# Autodesk Inventor assembly: 마지막센서
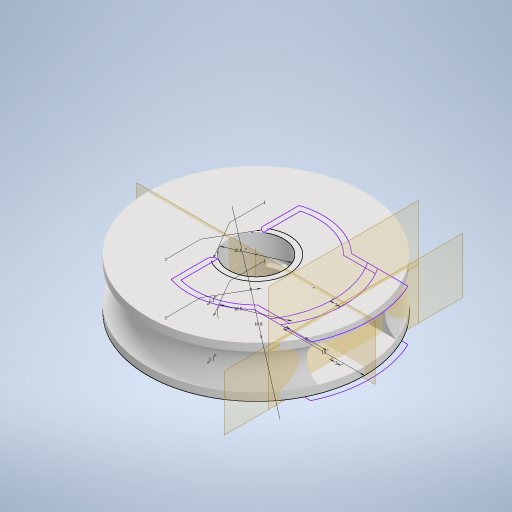
[picture p0: Inventor's stored thumbnail of the model, 512x512]
Saved by Autodesk Inventor 2023 (Build 270158000, 158)
## iProperties
Created: 2023-05-17
Part Number: 마지막센서
Document SubType Name: Assembly
Designer: rlatk
Author: rlatk
## Documents named in this file (3)
- C:\Users\rlatk\Desktop\코일건\코일건 부품\마지막센서.iam
- C:\Users\rlatk\Desktop\코일건\코일건 부품\마지막부품(꼽히는거).ipt
- C:\Users\rlatk\Desktop\코일건\코일건 부품\ir다이오드(마지막).ipt
## Components (3 placed, 2 different names)
1. 마지막부품(꼽히는거):1 — 회전:1, 각도:1, 접선:1, 회전:2
2. ir다이오드(마지막):1 — 회전:1
3. ir다이오드(마지막):2 — 회전:2
## Relationships (4: RevoluteJoint 2, Angle 1, Tangent 1)
- 회전:1 [RevoluteJoint]: 마지막부품(꼽히는거):1 ↔ ir다이오드(마지막):1
- 각도:1 [Angle] (0 deg): 마지막부품(꼽히는거):1
- 접선:1 [Tangent]: 마지막부품(꼽히는거):1
- 회전:2 [RevoluteJoint]: 마지막부품(꼽히는거):1 ↔ ir다이오드(마지막):2
